# Autodesk Inventor assembly: Assembly_Cube_VCA_v0
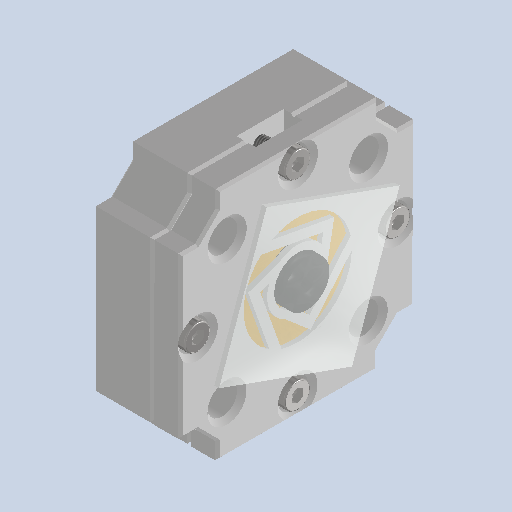
[picture p0: Inventor's stored thumbnail of the model, 512x512]
Saved by Autodesk Inventor 2022.3 (Build 263350000, 350)
## iProperties
Created: 2021-12-31
Part Number: Assembly_Cube_VCA_v0
Document SubType Name: Assembly
Designer: diederichbenedict
Mass: 22.6345 g
Surface Area: 191.935 cm^2
Volume: 22.6345 cm^3
Density: 1 g/cm^3
Author: diederichbenedict
## Documents named in this file (11)
- G:\My Drive\ASP - M.Sc. Photonics\Practical Modules\MODULE 4 - Master Thesis\2.Experiments\Modules\11.Reference_Mirror_Module\Reference_Mirror_with_UC2-VCA_Module\Assembly_Cube_VCA_v0.iam
- G:\My Drive\ASP - M.Sc. Photonics\Practical Modules\MODULE 4 - Master Thesis\2.Experiments\Modules\11.Reference_Mirror_Module\Reference_Mirror_with_UC2-VCA_Module\50_ETL_28by_coil.ipt
- G:\My Drive\ASP - M.Sc. Photonics\Practical Modules\MODULE 4 - Master Thesis\2.Experiments\Modules\11.Reference_Mirror_Module\Reference_Mirror_with_UC2-VCA_Module\00_Ringmagnet_10x5x3mm.ipt
- G:\My Drive\ASP - M.Sc. Photonics\Practical Modules\MODULE 4 - Master Thesis\2.Experiments\Modules\11.Reference_Mirror_Module\Reference_Mirror_with_UC2-VCA_Module\50_ETL_Lid_v0.ipt
- G:\My Drive\ASP - M.Sc. Photonics\Practical Modules\MODULE 4 - Master Thesis\2.Experiments\Modules\11.Reference_Mirror_Module\Reference_Mirror_with_UC2-VCA_Module\00_Mirror_30x30.ipt
- G:\My Drive\ASP - M.Sc. Photonics\Practical Modules\MODULE 4 - Master Thesis\2.Experiments\Modules\11.Reference_Mirror_Module\Reference_Mirror_with_UC2-VCA_Module\50_ETL_Spring_v0.ipt
- G:\My Drive\ASP - M.Sc. Photonics\Practical Modules\MODULE 4 - Master Thesis\2.Experiments\Modules\11.Reference_Mirror_Module\Reference_Mirror_with_UC2-VCA_Module\50_ETL_Motionpart1_v0.ipt
- G:\My Drive\ASP - M.Sc. Photonics\Practical Modules\MODULE 4 - Master Thesis\2.Experiments\Modules\11.Reference_Mirror_Module\Reference_Mirror_with_UC2-VCA_Module\50_Assembly_ETL_Mould.ipt
- G:\My Drive\ASP - M.Sc. Photonics\Practical Modules\MODULE 4 - Master Thesis\2.Experiments\Modules\11.Reference_Mirror_Module\Reference_Mirror_with_UC2-VCA_Module\20_Cube_Insert_VCA_base_lower_v0.ipt
- G:\My Drive\ASP - M.Sc. Photonics\Practical Modules\MODULE 4 - Master Thesis\2.Experiments\Modules\11.Reference_Mirror_Module\Reference_Mirror_with_UC2-VCA_Module\20_Cube_Insert_VCA_base_upper_v0.ipt
- C:\Users\bingoeleda\Documents\Inventor\Content Center Files\R2022\en-US\DIN 912\DIN 912 - M3 x 0.5 x 10 x 8.75.ipt
## Components (13 placed, 10 different names)
1. 00_Ringmagnet_10x5x3mm:1 — Einfügen:16
2. 50_ETL_Lid_v0:1
3. 00_Mirror_30x30:1 — Rigid:2
4. DIN 912 - replaced by DIN EN ISO 4762 M3 x 10:1 — Rotational:4
5. 50_Assembly_ETL_Mould:3
6. 50_ETL_Motionpart1_v0:1 — Einfügen:16, Rotational:1, Rigid:2
7. 20_Cube_Insert_VCA_base_upper_v0:1 — Passend:1, Winkel:1, Passend:6, Fluchtend:1, Rotational:1, Rotational:2, Rigid:1
8. 50_ETL_Spring_v0:4 — Passend:7, Winkel:2, Fluchtend:1
9. 50_ETL_28by_coil:1 — Rigid:1
10. 20_Cube_Insert_VCA_base_lower_v0:1 — Rotational:2, Rotational:4, Rotational:5, Rotational:6, Rotational:7
11. DIN 912 - replaced by DIN EN ISO 4762 M3 x 10:2 — Rotational:5
12. DIN 912 - replaced by DIN EN ISO 4762 M3 x 10:3 — Rotational:7
13. DIN 912 - replaced by DIN EN ISO 4762 M3 x 10:4 — Rotational:6
## Relationships (15: RevoluteJoint 6, Mate 3, Angle 2, WeldJoint 2, Flush 1, Insert 1)
- Passend:1 [Mate]: 20_Cube_Insert_VCA_base_upper_v0:1
- Winkel:1 [Angle] (0 deg): 20_Cube_Insert_VCA_base_upper_v0:1
- Passend:6 [Mate]: 20_Cube_Insert_VCA_base_upper_v0:1
- Passend:7 [Mate]: 50_ETL_Spring_v0:4
- Winkel:2 [Angle] (0 deg): 50_ETL_Spring_v0:4
- Fluchtend:1 [Flush]: 20_Cube_Insert_VCA_base_upper_v0:1 ↔ 50_ETL_Spring_v0:4
- Einfügen:16 [Insert] (3 mm): 00_Ringmagnet_10x5x3mm:1 ↔ 50_ETL_Motionpart1_v0:1
- Rotational:1 [RevoluteJoint]: 50_ETL_Motionpart1_v0:1 ↔ 20_Cube_Insert_VCA_base_upper_v0:1
- Rotational:2 [RevoluteJoint]: 20_Cube_Insert_VCA_base_upper_v0:1 ↔ 20_Cube_Insert_VCA_base_lower_v0:1
- Rigid:1 [WeldJoint]: 20_Cube_Insert_VCA_base_upper_v0:1 ↔ 50_ETL_28by_coil:1
- Rigid:2 [WeldJoint]: 00_Mirror_30x30:1 ↔ 50_ETL_Motionpart1_v0:1
- Rotational:4 [RevoluteJoint]: DIN 912 - replaced by DIN EN ISO 4762 M3 x 10:1 ↔ 20_Cube_Insert_VCA_base_lower_v0:1
- Rotational:5 [RevoluteJoint]: 20_Cube_Insert_VCA_base_lower_v0:1 ↔ DIN 912 - replaced by DIN EN ISO 4762 M3 x 10:2
- Rotational:6 [RevoluteJoint]: 20_Cube_Insert_VCA_base_lower_v0:1 ↔ DIN 912 - replaced by DIN EN ISO 4762 M3 x 10:4
- Rotational:7 [RevoluteJoint]: 20_Cube_Insert_VCA_base_lower_v0:1 ↔ DIN 912 - replaced by DIN EN ISO 4762 M3 x 10:3
